# Autodesk Inventor assembly: FrameCenterStructure
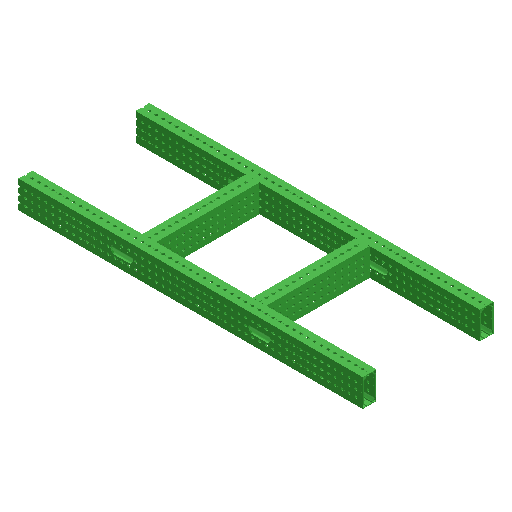
[picture p0: Inventor's stored thumbnail of the model, 512x512]
Saved by Autodesk Inventor 2023 (Build 270158000, 158)
## iProperties
Created: 2023-10-29
Part Number: FrameCenterStructure
Document SubType Name: Assembly
Designer: adamarnold
Author: adamarnold
## Documents named in this file (3)
- J:\My Drive\1939\2_Design\2023-2024\Swerve Test\Subassemblies\FrameCenterStructure.iam
- J:\My Drive\1939\2_Design\2023-2024\Parts\Cut Stock\2x1 Grid\Test_Swerve_Support_Grid.ipt
- J:\My Drive\1939\2_Design\2023-2024\Parts\Cut Stock\2x1 Grid\Battery_Grid.ipt
## Components (4 placed, 2 different names)
1. Test_Swerve_Support_Grid:1 — Flush:3, Mate:2, Flush:5, Flush:6, Flush:7
2. Test_Swerve_Support_Grid:2 — Mate:1, Mate:3, Flush:6, Flush:7
3. Battery_Grid:1 — Mate:1, Flush:2, Flush:5, Mate:4
4. Battery_Grid:2 — Flush:2, Flush:3, Mate:2, Mate:3, Mate:4
## Relationships (9: Flush 5, Mate 4)
- Mate:1: Test_Swerve_Support_Grid:2 ↔ Battery_Grid:1
- Flush:2: Battery_Grid:1 ↔ Battery_Grid:2
- Flush:3: Test_Swerve_Support_Grid:1 ↔ Battery_Grid:2
- Mate:2: Test_Swerve_Support_Grid:1 ↔ Battery_Grid:2
- Mate:3: Test_Swerve_Support_Grid:2 ↔ Battery_Grid:2
- Flush:5 (203.2 mm): Test_Swerve_Support_Grid:1 ↔ Battery_Grid:1
- Mate:4 (177.8 mm): Battery_Grid:1 ↔ Battery_Grid:2
- Flush:6: Test_Swerve_Support_Grid:1 ↔ Test_Swerve_Support_Grid:2
- Flush:7: Test_Swerve_Support_Grid:1 ↔ Test_Swerve_Support_Grid:2
